# Autodesk Inventor assembly: roll_support_front_v2
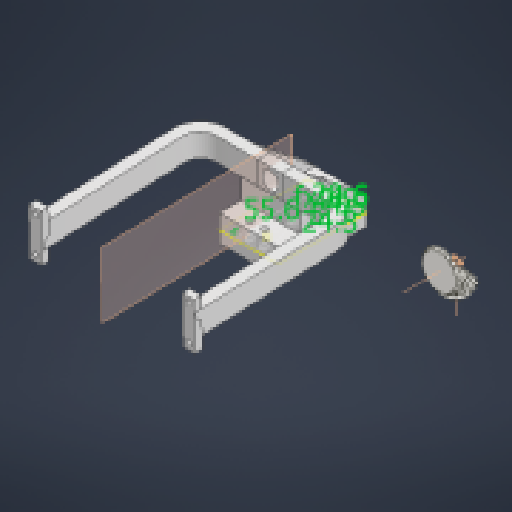
[picture p0: Inventor's stored thumbnail of the model, 512x512]
Saved by Autodesk Inventor 2026.1 (Build 301233020, 233B)
## iProperties
Created: 2025-11-28
Part Number: roll_support_front_v2
Document SubType Name: Assembly
Designer: jaewook
Author: jaewook
## Documents named in this file (6)
- C:\Users\kjh19\Documents\Inventor\project\final\roll_support_front_v2.iam
- C:\Users\kjh19\Documents\Inventor\project\proto2\example\솔리드7.ipt
- C:\Users\kjh19\Desktop\roll_motor\디자인 액셀러레이터\베벨 기어2.iam
- C:\Users\kjh19\Desktop\motor_clamp.ipt
- C:\Users\kjh19\Desktop\connector.ipt
- C:\Users\kjh19\Downloads\Servo+9imod+DS35MG-180\Servo-9imod-DS35MG-180.ipt
## Components (5 placed, 5 different names)
1. 솔리드7:2 — 메이트:3, 메이트:4, 메이트:7, 메이트:8
2. 베벨 기어:1 [sub-assembly] — 메이트:1, 메이트:2, 메이트:5, 메이트:6
3. motor_clamp:2 — 메이트:1, 메이트:2, 메이트:3, 메이트:4
4. connector:1 — 메이트:5, 메이트:6
5. Servo-9imod-DS35MG-180:1 — 메이트:7, 메이트:8
## Relationships (8: Mate 8)
- 메이트:1 [Mate]: 베벨 기어:1 ↔ motor_clamp:2
- 메이트:2 [Mate]: 베벨 기어:1 ↔ motor_clamp:2
- 메이트:3 [Mate]: 솔리드7:2 ↔ motor_clamp:2
- 메이트:4 [Mate]: 솔리드7:2 ↔ motor_clamp:2
- 메이트:5 [Mate]: 베벨 기어:1 ↔ connector:1
- 메이트:6 [Mate]: 베벨 기어:1 ↔ connector:1
- 메이트:7 [Mate]: 솔리드7:2 ↔ Servo-9imod-DS35MG-180:1
- 메이트:8 [Mate]: 솔리드7:2 ↔ Servo-9imod-DS35MG-180:1
